# Autodesk Inventor assembly: Print_Assembly
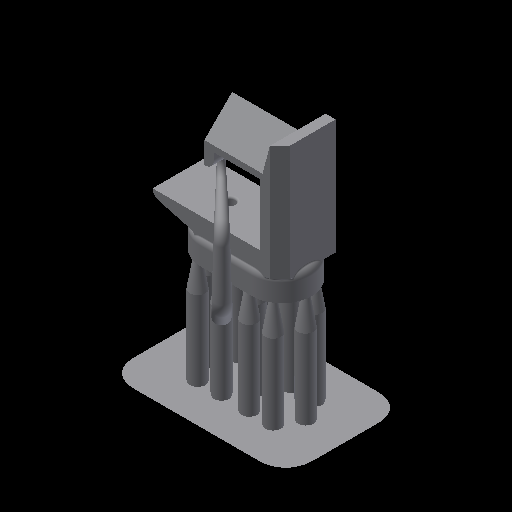
[picture p0: Inventor's stored thumbnail of the model, 512x512]
Saved by Autodesk Inventor 2026.2 (Build 302298010, 298A)
## iProperties
Manager: MANUTENÇÃO GUIFÕES - CP
Company: CP
Created: 2025-09-03
Part Number: Print_Assembly
Project: 0.00 0000/00
Checked By: PMFIGUEIREDO
Engr Approved By: JSSILVA
Description: NOME DA PEÇA/MONTAGEM
Document SubType Name: Assembly
Designer: TPMIRANDA
Engineer: ISO 2768 - m K
Authority: Nº DESENHO PELO QUAL FOI SUBSITUIDO
Stock Number: 00000-000
Title: UME 3400
Subject: CAIXA, INTERIOR, SUPORTE,
Author: TPMIRANDA
Keywords: Caixa de comentários. Substituir texto, ou eliminar.
Comments: UQE2300 UQE2400 UTE2240 UDD9630 CARRUAGENS SIMAFE CARRUAGENS CAF CARRUAGENS ARCO
Revision Number: Nº DESENHO QUE SUBSTITUI
## Documents named in this file (6)
- C:\Users\tpmiranda\OneDrive - Comboios de Portugal EPE\Engate CNMF\Montagem\Print_Assembly_N_Adapt_NEM356.iam
- C:\Users\tpmiranda\OneDrive - Comboios de Portugal EPE\Engate CNMF\Montagem\Stand.ipt
- C:\Users\tpmiranda\OneDrive - Comboios de Portugal EPE\Engate CNMF\Engates\Engate CNMF N Adapter\Engate CNMF PROFI-5.00.ipt
- C:\Users\tpmiranda\OneDrive - Comboios de Portugal EPE\Engate CNMF\Engates\Engate CNMF N Adapter.ipt
- C:\Users\tpmiranda\OneDrive - Comboios de Portugal EPE\Engate CNMF\Montagem\Stand_Branch_Short.ipt
- C:\Users\tpmiranda\OneDrive - Comboios de Portugal EPE\Engate CNMF\Montagem\Base N Wide.ipt
## Components (15 placed, 4 different names)
1. Base N Wide:1 — Alinhado:13, Alinhado:14, Coincidente:25, Coincidente:2, Coincidente:20
2. Stand_Branch_Short:2 — Coincidente:23, Coincidente:24
3. Stand_Branch_Short:1 — Coincidente:21, Coincidente:22
4. Engate CNMF PROFI-5.00:1 — Coincidente:1, Alinhado:16, Coincidente:3, Alinhado:17, Coincidente:4, Coincidente:19, Alinhado:18, Coincidente:22, Coincidente:24, Coincidente:25
5. Stand:1 — Coincidente:1, Coincidente:2, Alinhado:17, Coincidente:4
6. Stand:2 — Coincidente:19, Coincidente:20, Alinhado:18
7. Stand:3
8. Stand:4
9. Stand:9 — Coincidente:21
10. Stand:10 — Coincidente:23
11. Stand:6
12. Stand:7
13. Stand:8
14. Stand:11
15. Stand:12
## Component patterns: (2 elements), (5 elements, first: Stand:2), Component Pattern 12:2 (5 elements)
## Relationships (16: Mate 11, Flush 5)
- Alinhado:13 [Flush]: Base N Wide:1
- Alinhado:14 [Flush]: Base N Wide:1
- Coincidente:25 [Mate]: Base N Wide:1 ↔ Engate CNMF PROFI-5.00:1
- Coincidente:1 [Mate]: Engate CNMF PROFI-5.00:1 ↔ Stand:1
- Coincidente:2 [Mate]: Base N Wide:1 ↔ Stand:1
- Alinhado:16 [Flush]: Engate CNMF PROFI-5.00:1
- Coincidente:3 [Mate] (-3 mm): Engate CNMF PROFI-5.00:1
- Alinhado:17 [Flush]: Engate CNMF PROFI-5.00:1 ↔ Stand:1
- Coincidente:4 [Mate]: Engate CNMF PROFI-5.00:1 ↔ Stand:1
- Coincidente:19 [Mate]: Engate CNMF PROFI-5.00:1 ↔ Stand:2
- Coincidente:20 [Mate]: Base N Wide:1 ↔ Stand:2
- Alinhado:18 [Flush] (2.5 mm): Engate CNMF PROFI-5.00:1 ↔ Stand:2
- Coincidente:21 [Mate]: Stand_Branch_Short:1 ↔ Stand:9
- Coincidente:22 [Mate]: Stand_Branch_Short:1 ↔ Engate CNMF PROFI-5.00:1
- Coincidente:23 [Mate]: Stand_Branch_Short:2 ↔ Stand:10
- Coincidente:24 [Mate]: Stand_Branch_Short:2 ↔ Engate CNMF PROFI-5.00:1
